# Autodesk Inventor assembly: ASY APN 1440 FDS Top elbow
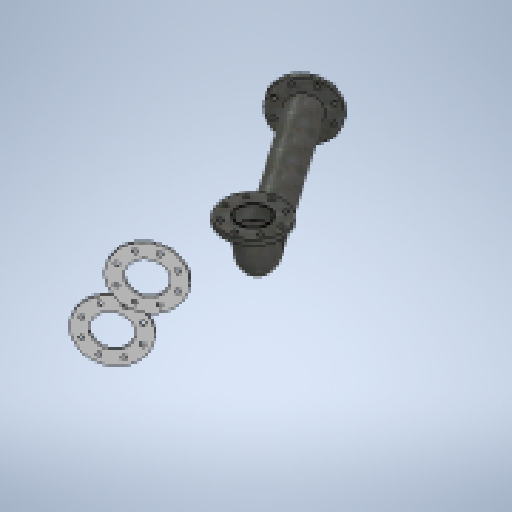
[picture p0: Inventor's stored thumbnail of the model, 512x512]
Saved by Autodesk Inventor 2025.3 (Build 293356030, 356C)
## iProperties
Created: 2025-07-10
Part Number: ASY APN 1440 FDS Top elbow
Document SubType Name: Assembly
Designer: user
Author: user
## Documents named in this file (6)
- C:\Users\admin\Yandex.Disk\home pc\Inventor\ANP--Antipayuta\ASY APN 1440 FDS Top elbow.iam
- C:\Users\admin\Yandex.Disk\home pc\Inventor\ANP--Antipayuta\DIN 2576 Slip-On Flange for Welding Series 1 (ISO) - PN 10 80 x 88.9.ipt
- C:\Users\admin\Yandex.Disk\home pc\Inventor\ANP--Antipayuta\APN 1442 FDS  tube 1.ipt
- C:\Users\admin\Yandex.Disk\home pc\Inventor\ANP--Antipayuta\APN 1441 FDS tube 1.ipt
- C:\Users\admin\Yandex.Disk\home pc\Inventor\ANP--Antipayuta\JIS B 2312 90 Deg Long Elbow Steel 100A x Sch 40.ipt
- C:\Users\admin\Yandex.Disk\home pc\Inventor\ANP--Antipayuta\APN 1433 FDS flange DN100.ipt
## Components (7 placed, 5 different names)
1. DIN 2576 Slip-On Flange for Welding Series 1 (ISO) - PN 10 80 x 88.9.ipt:1 — Rigid:7
2. APN 1441 FDS tube 1.ipt:1 — Rigid:7, Rotational:1
3. JIS B 2312 90 Deg Long Elbow Steel 100A x Sch 40.ipt:1
4. APN 1442 FDS  tube 1.ipt:1
5. DIN 2576 Slip-On Flange for Welding Series 1 (ISO) - PN 10 80 x 88.9.ipt:2 — Rotational:2
6. APN 1433 FDS flange DN100:1 — Rotational:1
7. APN 1433 FDS flange DN100:2 — Rotational:2
## Relationships (6: WeldJoint 4, RevoluteJoint 2)
- [WeldJoint]: APN 1441 FDS tube 1.ipt:1 ↔ JIS B 2312 90 Deg Long Elbow Steel 100A x Sch 40.ipt:1
- [WeldJoint]: JIS B 2312 90 Deg Long Elbow Steel 100A x Sch 40.ipt:1 ↔ APN 1442 FDS  tube 1.ipt:1
- [WeldJoint]: APN 1442 FDS  tube 1.ipt:1 ↔ DIN 2576 Slip-On Flange for Welding Series 1 (ISO) - PN 10 80 x 88.9.ipt:2
- Rigid:7 [WeldJoint]: DIN 2576 Slip-On Flange for Welding Series 1 (ISO) - PN 10 80 x 88.9.ipt:1 ↔ APN 1441 FDS tube 1.ipt:1
- Rotational:1 [RevoluteJoint]: APN 1441 FDS tube 1.ipt:1 ↔ APN 1433 FDS flange DN100:1
- Rotational:2 [RevoluteJoint]: DIN 2576 Slip-On Flange for Welding Series 1 (ISO) - PN 10 80 x 88.9.ipt:2 ↔ APN 1433 FDS flange DN100:2
